# Autodesk Inventor assembly: Сборка1
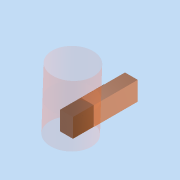
[picture p0: Inventor's stored thumbnail of the model, 180x180]
Saved by Autodesk Inventor 2019 (Build 230136000, 136)
## iProperties
Created: 2021-02-11
Part Number: Сборка1
Material: Типовые
Document SubType Name: Assembly
Designer: Kurbatova
Author: Kurbatova
## Documents named in this file (3)
- C:\Users\Kurbatova\source\LW2020\lw_2021\LW_SAPR\Сборки\Сборка1.iam
- C:\Users\Kurbatova\source\LW2020\lw_2021\LW_SAPR\Детали\Деталь2.ipt
- C:\Users\Kurbatova\source\LW2020\lw_2021\LW_SAPR\Детали\Деталь1.ipt
## Components (4 placed, 2 different names)
1. Деталь2:1 — Совмещение:1, Вставка:1
2. Деталь1:1 — Совмещение:1, Угол:1
3. Деталь2:2 — Вставка:1, Касательность:1
4. Деталь1:2 — Угол:1, Касательность:1
## Relationships (4: Mate 1, Insert 1, Angle 1, Tangent 1)
- Совмещение:1 [Mate]: Деталь2:1 ↔ Деталь1:1
- Вставка:1 [Insert]: Деталь2:1 ↔ Деталь2:2
- Угол:1 [Angle] (0 deg): Деталь1:1 ↔ Деталь1:2
- Касательность:1 [Tangent]: Деталь2:2 ↔ Деталь1:2
